# Autodesk Inventor assembly: Bodenplatte
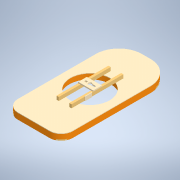
[picture p0: Inventor's stored thumbnail of the model, 180x180]
Saved by Autodesk Inventor 2020.3 (Build 243373010, 373A)
## iProperties
Created: 2021-01-31
Part Number: Bodenplatte
Document SubType Name: Assembly
Designer: Stefan
Author: Stefan
Title: Luftkissenboot-Bodenplatte
## Documents named in this file (8)
- D:\Stefan\Schule\HTL\Diplomarbeit\git\Inventor\Bodenplatte\Bodenplatte.iam
- D:\Stefan\Schule\HTL\Diplomarbeit\git\Inventor\Bodenplatte\Bodenplatte-Holz.ipt
- D:\Stefan\Schule\HTL\Diplomarbeit\git\Inventor\Bodenplatte\40x60Staffel.ipt
- D:\Stefan\Schule\HTL\Diplomarbeit\git\Inventor\Bodenplatte\MotorHalterung.ipt
- D:\Stefan\Schule\HTL\Diplomarbeit\git\Inventor\Bodenplatte\XPS.ipt
- D:\Stefan\Schule\HTL\Diplomarbeit\git\Inventor\Bodenplatte\HolzLatteLinks.ipt
- D:\Stefan\Schule\HTL\Diplomarbeit\git\Inventor\Bodenplatte\HolzPlatterechts.ipt
- D:\Stefan\Schule\HTL\Diplomarbeit\git\Inventor\Bodenplatte\HalterungMotorregler.ipt
## Components (9 placed, 7 different names)
1. Bodenplatte-Holz:1 — Passend:1, Passend:2, Passend:3, Passend:4, Passend:8, Fluchtend:4, Fluchtend:5
2. 40x60Staffel:1 — Passend:1, Passend:2, Passend:16, Fluchtend:6, Fluchtend:7, Passend:17, Fluchtend:8
3. 40x60Staffel:2 — Passend:3, Passend:4, Passend:15
4. MotorHalterung:1 — Passend:7, Fluchtend:2, Fluchtend:3, Passend:15, Passend:16, Fluchtend:6, Fluchtend:7
5. MotorHalterung:2 — Passend:7, Fluchtend:2, Fluchtend:3
6. XPS:1 — Passend:8, Fluchtend:4, Fluchtend:5, Passend:9, Passend:10, Passend:11, Passend:12, Passend:13, Passend:14
7. HolzLatteLinks:1 — Passend:9, Passend:10, Passend:11
8. HolzLatteRechts:1 — Passend:12, Passend:13, Passend:14
9. HalterungMotorregler:1 — Passend:17, Fluchtend:8
## Relationships (22: Mate 15, Flush 7)
- Passend:1 [Mate]: Bodenplatte-Holz:1 ↔ 40x60Staffel:1
- Passend:2 [Mate]: Bodenplatte-Holz:1 ↔ 40x60Staffel:1
- Passend:3 [Mate]: Bodenplatte-Holz:1 ↔ 40x60Staffel:2
- Passend:4 [Mate]: Bodenplatte-Holz:1 ↔ 40x60Staffel:2
- Passend:7 [Mate]: MotorHalterung:1 ↔ MotorHalterung:2
- Fluchtend:2 [Flush]: MotorHalterung:1 ↔ MotorHalterung:2
- Fluchtend:3 [Flush]: MotorHalterung:1 ↔ MotorHalterung:2
- Passend:8 [Mate]: Bodenplatte-Holz:1 ↔ XPS:1
- Fluchtend:4 [Flush]: Bodenplatte-Holz:1 ↔ XPS:1
- Fluchtend:5 [Flush]: Bodenplatte-Holz:1 ↔ XPS:1
- Passend:9 [Mate]: XPS:1 ↔ HolzLatteLinks:1
- Passend:10 [Mate]: XPS:1 ↔ HolzLatteLinks:1
- Passend:11 [Mate]: XPS:1 ↔ HolzLatteLinks:1
- Passend:12 [Mate]: XPS:1 ↔ HolzLatteRechts:1
- Passend:13 [Mate]: XPS:1 ↔ HolzLatteRechts:1
- Passend:14 [Mate]: XPS:1 ↔ HolzLatteRechts:1
- Passend:15 [Mate]: 40x60Staffel:2 ↔ MotorHalterung:1
- Passend:16 [Mate]: 40x60Staffel:1 ↔ MotorHalterung:1
- Fluchtend:6 [Flush]: 40x60Staffel:1 ↔ MotorHalterung:1
- Fluchtend:7 [Flush] (375 mm): 40x60Staffel:1 ↔ MotorHalterung:1
- Passend:17 [Mate]: 40x60Staffel:1 ↔ HalterungMotorregler:1
- Fluchtend:8 [Flush]: 40x60Staffel:1 ↔ HalterungMotorregler:1
